# Autodesk Inventor assembly: MotorRight
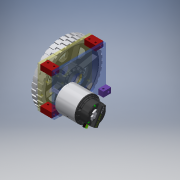
[picture p0: Inventor's stored thumbnail of the model, 180x180]
Saved by Autodesk Inventor 2019 (Build 230136000, 136)
## iProperties
Created: 2020-03-02
Part Number: MotorRight
Document SubType Name: Assembly
Designer: james
Author: james
## Documents named in this file (7)
- F:\JimsRobot\FIRSTRobots\Design\TornadoPlatypus\MotorRight.iam
- F:\JimsRobot\FIRSTRobots\Design\TornadoPlatypus\InsideMotorPlate.ipt
- F:\JimsRobot\FIRSTRobots\Design\Library\CTR\Falcon\217-6515 20191025.iam
- F:\JimsRobot\FIRSTRobots\Design\TornadoPlatypus\MotorSpacerBlock.ipt
- F:\JimsRobot\FIRSTRobots\Design\Library\AndyMark\6 HiGrip Asm Rev II.iam
- F:\JimsRobot\FIRSTRobots\Design\TornadoPlatypus\MotorSpacerBlock3.ipt
- F:\JimsRobot\FIRSTRobots\Design\TornadoPlatypus\OutsideMotorPlate.ipt
## Components (8 placed, 6 different names)
1. InsideMotorPlate:1 — Mate:1, Mate:2, Mate:3, Mate:4, Mate:6, Mate:7, Mate:8, Flush:1, Mate:9, Flush:2, Mate:11, Flush:4
2. 217-6515 20191025:1 [sub-assembly] — Mate:1, Mate:2, Mate:3
3. MotorSpacerBlock:1 — Mate:7, Mate:9, Flush:2, Mate:24, Mate:25
4. MotorSpacerBlock:2 — Mate:4, Mate:11, Flush:4
5. MotorSpacerBlock:3 — Mate:6, Mate:8, Flush:1, Mate:14
6. OutsideMotorPlate:2 — Mate:14, Mate:15, Mate:16, Mate:24, Mate:25
7. 6 HiGrip Asm Rev II:1 [sub-assembly] — Mate:15, Mate:16
8. MotorSpacerBlock3:1
## Relationships (17: Mate 14, Flush 3)
- Mate:1: InsideMotorPlate:1 ↔ 217-6515 20191025:1
- Mate:2: InsideMotorPlate:1 ↔ 217-6515 20191025:1
- Mate:3: InsideMotorPlate:1 ↔ 217-6515 20191025:1
- Mate:4: InsideMotorPlate:1 ↔ MotorSpacerBlock:2
- Mate:6: InsideMotorPlate:1 ↔ MotorSpacerBlock:3
- Mate:7: InsideMotorPlate:1 ↔ MotorSpacerBlock:1
- Mate:8: InsideMotorPlate:1 ↔ MotorSpacerBlock:3
- Flush:1: InsideMotorPlate:1 ↔ MotorSpacerBlock:3
- Mate:9: InsideMotorPlate:1 ↔ MotorSpacerBlock:1
- Flush:2: InsideMotorPlate:1 ↔ MotorSpacerBlock:1
- Mate:11: InsideMotorPlate:1 ↔ MotorSpacerBlock:2
- Flush:4: InsideMotorPlate:1 ↔ MotorSpacerBlock:2
- Mate:14: MotorSpacerBlock:3 ↔ OutsideMotorPlate:2
- Mate:15: OutsideMotorPlate:2 ↔ 6 HiGrip Asm Rev II:1
- Mate:16: OutsideMotorPlate:2 ↔ 6 HiGrip Asm Rev II:1
- Mate:24: MotorSpacerBlock:1 ↔ OutsideMotorPlate:2
- Mate:25: MotorSpacerBlock:1 ↔ OutsideMotorPlate:2
